# Autodesk Inventor assembly: Baugruppe1
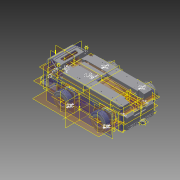
[picture p0: Inventor's stored thumbnail of the model, 180x180]
Saved by Autodesk Inventor 2015 (Build 190159000, 159)
## iProperties
Created: 2018-11-29
Part Number: Baugruppe1
Document SubType Name: Assembly
Designer: Boris
Author: Boris
## Documents named in this file (20)
- D:\Wisag Hiserv\HiSERV Smart Drive\WorkOrder\3D - Teile\Baugruppe1.iam
- D:\Wisag Hiserv\HiSERV Smart Drive\WorkOrder\3D - Teile\Chassis.ipt
- D:\Wisag Hiserv\HiSERV Smart Drive\WorkOrder\3D - Teile\ChassisLinksUnten.ipt
- D:\Wisag Hiserv\HiSERV Smart Drive\WorkOrder\3D - Teile\ChassisHintenUnten.ipt
- D:\Wisag Hiserv\HiSERV Smart Drive\WorkOrder\3D - Teile\ChassisRechtsUnten.ipt
- D:\Wisag Hiserv\HiSERV Smart Drive\WorkOrder\3D - Teile\ChassisRechtsUntenKlappe.ipt
- D:\Wisag Hiserv\HiSERV Smart Drive\WorkOrder\3D - Teile\SchleppstangeHauptTeil.ipt
- D:\Wisag Hiserv\HiSERV Smart Drive\WorkOrder\3D - Teile\KabineChassis.iam
- D:\Wisag Hiserv\HiSERV Smart Drive\WorkOrder\3D - Teile\KarosserieDachTeil1.ipt
- D:\Wisag Hiserv\HiSERV Smart Drive\WorkOrder\3D - Teile\KarosserieDachTeil2.ipt
- D:\Wisag Hiserv\HiSERV Smart Drive\WorkOrder\3D - Teile\KarosserieDachTeil3.ipt
- D:\Wisag Hiserv\HiSERV Smart Drive\WorkOrder\3D - Teile\ChassisOberTeil.ipt
- D:\Wisag Hiserv\HiSERV Smart Drive\WorkOrder\3D - Teile\LenkungStütze.ipt
- D:\Wisag Hiserv\HiSERV Smart Drive\WorkOrder\3D - Teile\LenkungTeil1.ipt
- D:\Wisag Hiserv\HiSERV Smart Drive\WorkOrder\3D - Teile\KugelLager.ipt
- D:\Wisag Hiserv\HiSERV Smart Drive\WorkOrder\3D - Teile\Rad_Axe_GummiVorne.iam
- D:\Wisag Hiserv\HiSERV Smart Drive\WorkOrder\3D - Teile\Sirene.ipt
- D:\Wisag Hiserv\HiSERV Smart Drive\WorkOrder\3D - Teile\KarosserieDachTeil3_MIR.ipt
- D:\Wisag Hiserv\HiSERV Smart Drive\WorkOrder\3D - Teile\KabineTürLinksRechts_MIR.ipt
- D:\Wisag Hiserv\HiSERV Smart Drive\WorkOrder\3D - Teile\KabineTürLinksRechts_MIR_MIR.ipt
## Components (32 placed, 19 different names)
1. Chassis:1 — Einfügen:1, Einfügen:2, Passend:1, Passend:2, Einfügen:5, Einfügen:10, Einfügen:11, Einfügen:12, Einfügen:13, Einfügen:14, Einfügen:15, Einfügen:17, Einfügen:19
2. ChassisLinksUnten:1 — Einfügen:1, Einfügen:6, Einfügen:9
3. ChassisHintenUnten:1 — Einfügen:2, Passend:1, Fluchtend:1, Passend:3, Passend:4
4. ChassisRechtsUnten:1 — Passend:2, Einfügen:3, Drehung:1, Einfügen:4
5. ChassisRechtsUntenKlappe:1 — Einfügen:3, Drehung:1, Einfügen:4
6. SchleppstangeHauptTeil:1 — Passend:4
7. KabineChassis:1 [sub-assembly] — Einfügen:5, Einfügen:21, Einfügen:22
8. KarosserieDachTeil1:1 — Einfügen:6, Einfügen:7, Einfügen:8
9. KarosserieDachTeil2:1 — Einfügen:7, Einfügen:8
10. KarosserieDachTeil3:1 — Einfügen:9, Passend:3
11. ChassisOberTeil:1 — Einfügen:16, Einfügen:18, Einfügen:20
12. LenkungStütze:1 — Einfügen:11, Einfügen:16
13. LenkungTeil1:1 — Symmetrie:1
14. LenkungStütze:2 — Einfügen:15
15. LenkungTeil1:2 — Symmetrie:1
16. LenkungStütze:3 — Einfügen:14
17. LenkungStütze:4 — Einfügen:13
18. LenkungStütze:5 — Einfügen:12
19. LenkungStütze:6 — Einfügen:10
20. KugelLager:1 — Einfügen:17
21. KugelLager:2 — Einfügen:20
22. KugelLager:3 — Einfügen:18
23. KugelLager:4 — Einfügen:19
24. Rad_Axe_GummiVorne:1 [sub-assembly]
25. Rad_Axe_GummiVorne:2 [sub-assembly]
26. Rad_Axe_GummiVorne:3 [sub-assembly]
27. Rad_Axe_GummiVorne:4 [sub-assembly]
28. Sirene:1 — Einfügen:21
29. Sirene:2 — Einfügen:22
30. KarosserieDachTeil3_MIR:1
31. KabineTürLinksRechts_MIR:1
32. KabineTürLinksRechts_MIR_MIR:1
## Relationships (29: Insert 22, Mate 4, RelateRotation 1, Flush 1, Symmetry 1)
- Einfügen:1 [Insert] (4 mm): Chassis:1 ↔ ChassisLinksUnten:1
- Einfügen:2 [Insert] (-3 mm): Chassis:1 ↔ ChassisHintenUnten:1
- Passend:1 [Mate]: Chassis:1 ↔ ChassisHintenUnten:1
- Passend:2 [Mate]: Chassis:1 ↔ ChassisRechtsUnten:1
- Einfügen:3 [Insert] (-5.5 mm): ChassisRechtsUnten:1 ↔ ChassisRechtsUntenKlappe:1
- Drehung:1 [RelateRotation] (1 ul): ChassisRechtsUnten:1 ↔ ChassisRechtsUntenKlappe:1
- Einfügen:4 [Insert]: ChassisRechtsUnten:1 ↔ ChassisRechtsUntenKlappe:1
- Einfügen:5 [Insert] (4 mm): Chassis:1 ↔ KabineChassis:1
- Einfügen:6 [Insert] (-4 mm): ChassisLinksUnten:1 ↔ KarosserieDachTeil1:1
- Fluchtend:1 [Flush]: ChassisHintenUnten:1
- Einfügen:7 [Insert]: KarosserieDachTeil1:1 ↔ KarosserieDachTeil2:1
- Einfügen:8 [Insert]: KarosserieDachTeil1:1 ↔ KarosserieDachTeil2:1
- Einfügen:9 [Insert]: ChassisLinksUnten:1 ↔ KarosserieDachTeil3:1
- Passend:3 [Mate]: ChassisHintenUnten:1 ↔ KarosserieDachTeil3:1
- Einfügen:10 [Insert]: Chassis:1 ↔ LenkungStütze:6
- Einfügen:11 [Insert]: Chassis:1 ↔ LenkungStütze:1
- Einfügen:12 [Insert]: Chassis:1 ↔ LenkungStütze:5
- Einfügen:13 [Insert]: Chassis:1 ↔ LenkungStütze:4
- Einfügen:14 [Insert]: Chassis:1 ↔ LenkungStütze:3
- Einfügen:15 [Insert]: Chassis:1 ↔ LenkungStütze:2
- Einfügen:16 [Insert]: ChassisOberTeil:1 ↔ LenkungStütze:1
- Einfügen:17 [Insert] (-4 mm): Chassis:1 ↔ KugelLager:1
- Einfügen:18 [Insert] (-4 mm): ChassisOberTeil:1 ↔ KugelLager:3
- Einfügen:19 [Insert] (-4 mm): Chassis:1 ↔ KugelLager:4
- Einfügen:20 [Insert] (-4 mm): ChassisOberTeil:1 ↔ KugelLager:2
- Symmetrie:1: LenkungTeil1:1 ↔ LenkungTeil1:2
- Einfügen:21 [Insert] (5 mm): KabineChassis:1 ↔ Sirene:1
- Einfügen:22 [Insert] (10 mm): KabineChassis:1 ↔ Sirene:2
- Passend:4 [Mate] (10 mm): ChassisHintenUnten:1 ↔ SchleppstangeHauptTeil:1
